# Autodesk Inventor assembly: Сборка_крепления_камеры
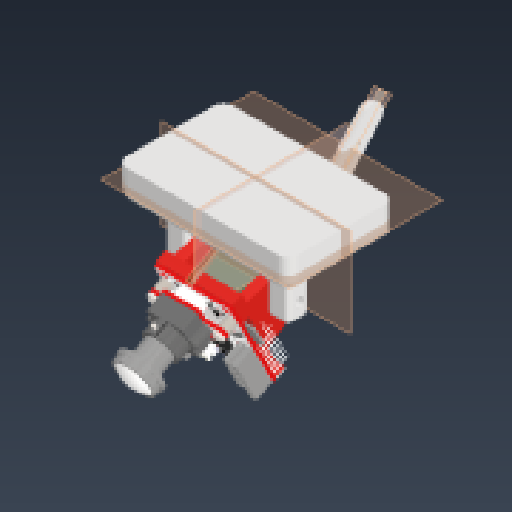
[picture p0: Inventor's stored thumbnail of the model, 512x512]
Saved by Autodesk Inventor 2023.2 (Build 272271030, 271C)
## iProperties
Created: 2025-10-07
Part Number: Сборка_крепления_камеры
Document SubType Name: Assembly
Designer: Олег Коноваленко
Author: Олег Коноваленко
## Documents named in this file (5)
- D:\!Rover\Rover\Rover_construction\Сборка_крепления_камеры.iam
- D:\!Rover\Rover\Rover_construction\Крепление_камеры.ipt
- D:\!Rover\Rover\Rover_construction\Качель камеры.ipt
- D:\!Rover\Rover\Rover_construction\openMV_H7\openmv4_h7\openmv4_h7.ipt
- D:\!Rover\Rover\Rover_construction\Качалка_крепления_камеры.ipt
## Components (4 placed, 4 different names)
1. Крепление_камеры:1 — Заподлицо:1, Цилиндрический:1, Касательность:1
2. Качель камеры:1 — Заподлицо:1, Цилиндрический:1, Совмещение:1, Заподлицо:2, Заподлицо:3, Заподлицо:4, С поворотом:1
3. openmv4_h7:1 — Совмещение:1, Заподлицо:2, Заподлицо:3
4. Качалка_крепления_камеры:1 — Заподлицо:4, С поворотом:1, Касательность:1
## Relationships (8: Flush 4, CylindricalJoint 1, Mate 1, RevoluteJoint 1, Tangent 1)
- Заподлицо:1 [Flush]: Крепление_камеры:1 ↔ Качель камеры:1
- Цилиндрический:1 [CylindricalJoint]: Крепление_камеры:1 ↔ Качель камеры:1
- Совмещение:1 [Mate]: Качель камеры:1 ↔ openmv4_h7:1
- Заподлицо:2 [Flush]: Качель камеры:1 ↔ openmv4_h7:1
- Заподлицо:3 [Flush]: Качель камеры:1 ↔ openmv4_h7:1
- Заподлицо:4 [Flush]: Качель камеры:1 ↔ Качалка_крепления_камеры:1
- С поворотом:1 [RevoluteJoint] (0.5 mm): Качель камеры:1 ↔ Качалка_крепления_камеры:1
- Касательность:1 [Tangent]: Крепление_камеры:1 ↔ Качалка_крепления_камеры:1
